# Autodesk Inventor assembly: Assembly
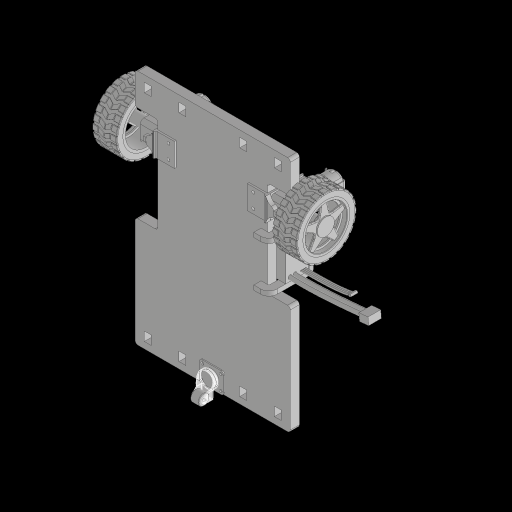
[picture p0: Inventor's stored thumbnail of the model, 512x512]
Saved by Autodesk Inventor 2024.3 (Build 283343010, 343A)
## iProperties
Created: 2025-04-09
Part Number: Assembly
Document SubType Name: Assembly
Designer: Oleg Kelner
Author: Oleg Kelner
## Documents named in this file (11)
- D:\Study\Prototyping\Prototyping-SS25-Team-C4\3DModels\Assembly.iam
- D:\Study\Prototyping\Prototyping-SS25-Team-C4\3DModels\Basic components\chassis.ipt
- D:\Study\Prototyping\Prototyping-SS25-Team-C4\3DModels\Basic components\motor-with-tire.ipt
- D:\Study\Prototyping\Prototyping-SS25-Team-C4\3DModels\Basic components\front-wheel.ipt
- D:\Study\Prototyping\Prototyping-SS25-Team-C4\3DModels\Basic components\motor-with-tire_MIR.ipt
- D:\Study\Prototyping\Prototyping-SS25-Team-C4\3DModels\Basic components\lipo-battery.ipt
- D:\Study\Prototyping\Prototyping-SS25-Team-C4\3DModels\Basic components\arduino.ipt
- D:\Study\Prototyping\Prototyping-SS25-Team-C4\3DModels\Basic components\breadboard.ipt
- D:\Study\Prototyping\Prototyping-SS25-Team-C4\3DModels\Basic components\motorcontroler.ipt
- D:\Study\Prototyping\Prototyping-SS25-Team-C4\3DModels\Oleg's details\vertMotorHolder.ipt
- D:\Study\Prototyping\Prototyping-SS25-Team-C4\3DModels\Oleg's details\batteryHolder.ipt
## Components (11 placed, 10 different names)
1. chassis:1 — Rigid:1, Rigid:2, Rigid:3, Slider:1
2. motor-with-tire:1 — Rotational:1, Rotational:2
3. front-wheel:1 — Rigid:1
4. motor-with-tire_MIR:1 — Rotational:3, Rotational:4
5. lipo-battery:1 — Slider:1, Slider:2
6. arduino:1
7. breadboard:1
8. motorcontroler:1
9. vertMotorHolder:1 — Rotational:1, Rotational:2, Rigid:3
10. vertMotorHolder:2 — Rotational:3, Rotational:4, Rigid:2
11. batteryHolder:1 — Slider:2
## Relationships (9: RevoluteJoint 4, WeldJoint 3, TranslationJoint 2)
- Rigid:1 [WeldJoint]: chassis:1 ↔ front-wheel:1
- Rotational:1 [RevoluteJoint]: motor-with-tire:1 ↔ vertMotorHolder:1
- Rotational:2 [RevoluteJoint]: motor-with-tire:1 ↔ vertMotorHolder:1
- Rotational:3 [RevoluteJoint]: motor-with-tire_MIR:1 ↔ vertMotorHolder:2
- Rotational:4 [RevoluteJoint]: motor-with-tire_MIR:1 ↔ vertMotorHolder:2
- Rigid:2 [WeldJoint] (-30 mm): chassis:1 ↔ vertMotorHolder:2
- Rigid:3 [WeldJoint] (30 mm): chassis:1 ↔ vertMotorHolder:1
- Slider:1 [TranslationJoint]: chassis:1 ↔ lipo-battery:1
- Slider:2 [TranslationJoint] (0.5 mm): lipo-battery:1 ↔ batteryHolder:1
